# Autodesk Inventor assembly: drives connected
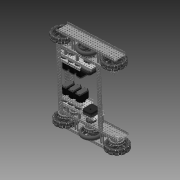
[picture p0: Inventor's stored thumbnail of the model, 180x180]
Saved by Autodesk Inventor 2014 SP1 (Build 180222100, 222)
## iProperties
Created: 2013-09-09
Part Number: drives connected
Document SubType Name: Assembly
Designer: Ryan
Sending System: SolidWorks 2013
Last Author: Ryan
Author: Ryan
## Documents named in this file (6)
- C:\Users\Ryan\Desktop\sw\toss up 1st A bot\inventor drive\drives connected.iam
- C:\Users\Ryan\Desktop\sw\toss up 1st A bot\inventor drive\one side of drive.iam
- C:\Users\Ryan\Desktop\sw\lib\Aperture VEX CAD Library\Hardware\8-32\8-32_.375.ipt
- C:\Users\Ryan\Desktop\sw\toss up 1st A bot\inventor drive\manual shifter and A bot gearbox.iam
- C:\Users\Ryan\Desktop\sw\lib\Aperture VEX CAD Library\Metal\L Bar\2 x 25.ipt
- C:\Users\Ryan\Desktop\sw\toss up 1st A bot\inventor drive\manual shifter and A bot gearbox_MIR.iam
## Components (12 placed, 5 different names)
1. 2 x 25:1 — Mate:1, Flush:2, Flush:3, Mate:3, Mate:5
2. 8-32_-375:21 — Mate:13, Mate:14, Mate:15
3. 8-32_-375:2 — Mate:16, Mate:17, Mate:18
4. 8-32_-375:22 — Mate:4, Mate:6, Mate:7
5. 8-32_-375:23 — Mate:8, Mate:9, Mate:10
6. 2 x 25:2 — Mate:11, Flush:7, Flush:8, Mate:20, Flush:14, Flush:15
7. 2 x 25:3 — Flush:2, Flush:3, Flush:4, Flush:5, Mate:5, Mate:7, Mate:8, Mate:9, Mate:10, Mate:13, Mate:14, Mate:15, Mate:16, Mate:17, Mate:18, Flush:13
8. 2 x 25:4 — Mate:12, Flush:9, Flush:12
9. one side of drive:1 [sub-assembly] — Mate:1, Flush:4, Flush:5, Mate:3, Mate:4, Mate:6, Mate:11, Flush:7, Flush:8, Mate:12, Flush:9, Mate:19, Flush:10, Flush:11, Flush:12
10. manual shifter and A bot gearbox:1 [sub-assembly] — Mate:19, Flush:10, Flush:11
11. one side of drive:2 [sub-assembly] — Mate:20, Flush:14, Flush:15
12. manual shifter and A bot gearbox_MIR:1 [sub-assembly]
## Relationships (32: Mate 19, Flush 13)
- Mate:1: 2 x 25:1 ↔ one side of drive:1
- Flush:2: 2 x 25:1 ↔ 2 x 25:3
- Flush:3: 2 x 25:1 ↔ 2 x 25:3
- Flush:4: 2 x 25:3 ↔ one side of drive:1
- Flush:5: 2 x 25:3 ↔ one side of drive:1
- Mate:3: 2 x 25:1 ↔ one side of drive:1
- Mate:4 (2.3114 mm): 8-32_-375:22 ↔ one side of drive:1
- Mate:5: 2 x 25:1 ↔ 2 x 25:3
- Mate:6 (2.3114 mm): 8-32_-375:22 ↔ one side of drive:1
- Mate:7: 8-32_-375:22 ↔ 2 x 25:3
- Mate:8 (2.3114 mm): 8-32_-375:23 ↔ 2 x 25:3
- Mate:9 (2.3114 mm): 8-32_-375:23 ↔ 2 x 25:3
- Mate:10: 8-32_-375:23 ↔ 2 x 25:3
- Mate:11: 2 x 25:2 ↔ one side of drive:1
- Flush:7: 2 x 25:2 ↔ one side of drive:1
- Flush:8: 2 x 25:2 ↔ one side of drive:1
- Mate:12: 2 x 25:4 ↔ one side of drive:1
- Flush:9: 2 x 25:4 ↔ one side of drive:1
- Mate:13 (2.3114 mm): 8-32_-375:21 ↔ 2 x 25:3
- Mate:14: 8-32_-375:21 ↔ 2 x 25:3
- Mate:15 (2.3114 mm): 8-32_-375:21 ↔ 2 x 25:3
- Mate:16 (2.3114 mm): 8-32_-375:2 ↔ 2 x 25:3
- Mate:17 (2.3114 mm): 8-32_-375:2 ↔ 2 x 25:3
- Mate:18: 8-32_-375:2 ↔ 2 x 25:3
- Mate:19: one side of drive:1 ↔ manual shifter and A bot gearbox:1
- Flush:10: one side of drive:1 ↔ manual shifter and A bot gearbox:1
- Flush:11: one side of drive:1 ↔ manual shifter and A bot gearbox:1
- Flush:12: 2 x 25:4 ↔ one side of drive:1
- Flush:13 (-158.75 mm): 2 x 25:3
- Mate:20: 2 x 25:2 ↔ one side of drive:2
- Flush:14: 2 x 25:2 ↔ one side of drive:2
- Flush:15: 2 x 25:2 ↔ one side of drive:2
## Named parameters: q = 2.3114 mm
